# Autodesk Inventor assembly: Hallmesssonde_finaleBaugruppe
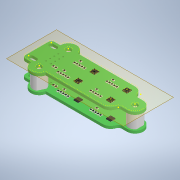
[picture p0: Inventor's stored thumbnail of the model, 180x180]
Saved by Autodesk Inventor 2022.2 (Build 262287010, 287A)
## iProperties
Created: 2024-01-10
Part Number: Hallmesssonde_finaleBaugruppe
Document SubType Name: Assembly
Designer: ppovolni
Author: ppovolni
## Documents named in this file (3)
- D:\3_Local_Projekte\_PaperGitHub\MiniBumblebee_LowFieldMapping\1_HallSensor\11_Hardware\112_CAD Files\SensorHead\SensorHead_ASM.iam
- D:\3_Local_Projekte\_PaperGitHub\MiniBumblebee_LowFieldMapping\1_HallSensor\11_Hardware\112_CAD Files\SensorHead\SensorHead_PCB_Single.ipt
- D:\3_Local_Projekte\_PaperGitHub\MiniBumblebee_LowFieldMapping\1_HallSensor\11_Hardware\112_CAD Files\SensorHead\Hallsensor_DistanceBolt_8mm4.ipt
## Components (5 placed, 2 different names)
1. Hallsensor_DistanceBolt_8mm4:1 — Passend:1, Passend:2
2. Hallsensor_DistanceBolt_8mm4:2 — Passend:3, Passend:6
3. Hallsensor_DistanceBolt_8mm4:3 — Passend:4, Passend:5
4. SensorHead_PCB_Single:1 — Passend:1, Passend:2, Passend:3, Passend:4, Passend:5, Passend:6, Fluchtend:1
5. SensorHead_PCB_Single:2
## Component patterns: (2 elements, first: SensorHead_PCB_Single:1)
## Relationships (7: Mate 6, Flush 1)
- Passend:1 [Mate]: Hallsensor_DistanceBolt_8mm4:1 ↔ SensorHead_PCB_Single:1
- Passend:2 [Mate]: Hallsensor_DistanceBolt_8mm4:1 ↔ SensorHead_PCB_Single:1
- Passend:3 [Mate]: Hallsensor_DistanceBolt_8mm4:2 ↔ SensorHead_PCB_Single:1
- Passend:4 [Mate]: Hallsensor_DistanceBolt_8mm4:3 ↔ SensorHead_PCB_Single:1
- Passend:5 [Mate]: Hallsensor_DistanceBolt_8mm4:3 ↔ SensorHead_PCB_Single:1
- Passend:6 [Mate]: Hallsensor_DistanceBolt_8mm4:2 ↔ SensorHead_PCB_Single:1
- Fluchtend:1 [Flush]: SensorHead_PCB_Single:1
